# Autodesk Inventor assembly: 3 Stage HD - CIM Sport
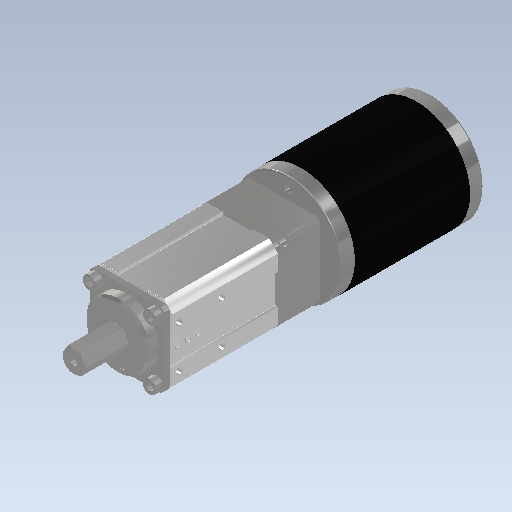
[picture p0: Inventor's stored thumbnail of the model, 512x512]
Saved by Autodesk Inventor 2020 (Build 240168000, 168)
## iProperties
Created: 2017-11-21
Part Number: 3 Stage HD - CIM Sport
Description: STEP AP203
Document SubType Name: Assembly
Designer: 1cikaychapman
Sending System: SolidWorks 2017
Preprocessor: SwSTEP 2.0
Title: am-3764 - 64_1 - CIM Sport.STEP
Revision Number: ANY
## Documents named in this file (11)
- C:\Users\autum\Google Drive\Iron Riders 4180 (Roosevelt Robotics)\2019-2020\Build_Design\Robot 2020 (1)\Climber\3 Stage HD - CIM Sport.iam
- C:\Users\autum\Google Drive\Iron Riders 4180 (Roosevelt Robotics)\2019-2020\Build_Design\Robot 2020 (1)\Climber\am-XXXX - 57 Sport 500 Hex Output Plug.iam
- C:\Users\autum\Google Drive\Iron Riders 4180 (Roosevelt Robotics)\2019-2020\Build_Design\Robot 2020 (1)\Climber\4_1 HD Output Stage.iam
- C:\Users\autum\Google Drive\Iron Riders 4180 (Roosevelt Robotics)\2019-2020\Build_Design\Robot 2020 (1)\Climber\am-XXXX - 4_1 Stage Long Sun Gear.iam
- C:\Users\autum\Google Drive\Iron Riders 4180 (Roosevelt Robotics)\2019-2020\Build_Design\Robot 2020 (1)\Climber\am-XXXX - 4_1 Stage.iam
- C:\Users\autum\Google Drive\Iron Riders 4180 (Roosevelt Robotics)\2019-2020\Build_Design\Robot 2020 (1)\Climber\am-XXXX - 57 Sport 3 Stage Ring Gear Housing.ipt
- C:\Users\autum\Google Drive\Iron Riders 4180 (Roosevelt Robotics)\2019-2020\Build_Design\Robot 2020 (1)\Climber\Thrust washer - 775 Sport.ipt
- C:\Users\autum\Google Drive\Iron Riders 4180 (Roosevelt Robotics)\2019-2020\Build_Design\Robot 2020 (1)\Climber\Cim Sport Motor Block.ipt
- C:\Users\autum\Google Drive\Iron Riders 4180 (Roosevelt Robotics)\2019-2020\Build_Design\Robot 2020 (1)\Climber\10-32 x 3.000 SHCS_90128A969.ipt
- C:\Users\autum\Google Drive\Iron Riders 4180 (Roosevelt Robotics)\2019-2020\Build_Design\Robot 2020 (1)\Climber\10-32 X 375 SHCS_90128A940.ipt
- C:\Users\autum\Google Drive\Iron Riders 4180 (Roosevelt Robotics)\2019-2020\Build_Design\Robot 2020 (1)\Climber\Mini_CIM_Motor_217-3371.ipt
## Components (12 placed, 12 different names)
1. am-XXXX - 57 Sport 500 Hex Output Plug_1 [sub-assembly]
2. 4_1 HD Output Stage_2 [sub-assembly]
3. am-XXXX - 4_1 Stage Long Sun Gear_3 [sub-assembly]
4. am-XXXX - 4_1 Stage_4 [sub-assembly]
5. am-XXXX - 57 Sport 3 Stage Ring Gear Housing_5
6. Thrust washer - 775 Sport_6
7. Cim Sport Motor Block_7 — Insert:1
8. 10-32 x 3.000 SHCS_90128A969_8
9. 10-32 x 3.000 SHCS_90128A969_9
10. 10-32 X 375 SHCS_90128A940_10
11. 10-32 X 375 SHCS_90128A940_11
12. Mini_CIM_Motor_217-3371:1 — Insert:1
## Relationships (1: Insert 1)
- Insert:1 (-33.02 mm): Cim Sport Motor Block_7 ↔ Mini_CIM_Motor_217-3371:1
